# Autodesk Inventor assembly: 24 Pin Straight Header
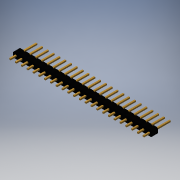
[picture p0: Inventor's stored thumbnail of the model, 180x180]
Saved by Autodesk Inventor 2016 (Build 200138000, 138)
## iProperties
Created: 2016-01-25
Part Number: 24 Pin Straight Header
Document SubType Name: Assembly
Designer: JLJ
Author: JLJ
## Documents named in this file (3)
- C:\Users\larra\Documents\GitHub\AirDataComputer\AirDataComputer\Hardware\3D support\teensy3.6\24 Pin Straight Header.iam
- 24 Pin Straight Header.iam
- C:\Users\larra\Documents\GitHub\AirDataComputer\AirDataComputer\Hardware\3D support\teensy3.6\Single Header Pin.iam
## Components (24 placed, 1 different names)
1. Single Header Pin:1 [sub-assembly] — Mate:1, Mate:2, Flush:1
2. Single Header Pin:2 [sub-assembly]
3. Single Header Pin:3 [sub-assembly]
4. Single Header Pin:4 [sub-assembly]
5. Single Header Pin:5 [sub-assembly]
6. Single Header Pin:6 [sub-assembly]
7. Single Header Pin:7 [sub-assembly]
8. Single Header Pin:8 [sub-assembly]
9. Single Header Pin:9 [sub-assembly]
10. Single Header Pin:10 [sub-assembly]
11. Single Header Pin:11 [sub-assembly]
12. Single Header Pin:12 [sub-assembly]
13. Single Header Pin:13 [sub-assembly]
14. Single Header Pin:14 [sub-assembly]
15. Single Header Pin:15 [sub-assembly]
16. Single Header Pin:16 [sub-assembly]
17. Single Header Pin:17 [sub-assembly]
18. Single Header Pin:18 [sub-assembly]
19. Single Header Pin:19 [sub-assembly]
20. Single Header Pin:20 [sub-assembly]
21. Single Header Pin:21 [sub-assembly]
22. Single Header Pin:22 [sub-assembly]
23. Single Header Pin:23 [sub-assembly]
24. Single Header Pin:24 [sub-assembly]
## Component patterns: (24 elements, first: Single Header Pin:1)
## Relationships (3: Mate 2, Flush 1)
- Mate:1: Single Header Pin:1
- Mate:2: Single Header Pin:1
- Flush:1: Single Header Pin:1
